# Autodesk Inventor assembly: Assembly Proximity Servo
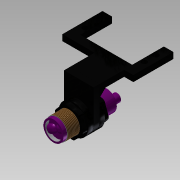
[picture p0: Inventor's stored thumbnail of the model, 180x180]
Saved by Autodesk Inventor 2015 SP1 (Build 190203100, 203)
## iProperties
Created: 2015-02-11
Part Number: Assembly Proximity Servo
Document SubType Name: Assembly
Designer: Rafi Kurnia Putra
Author: Rafi Kurnia Putra
## Documents named in this file (4)
- D:\Dropbox\krpai berkaki trui 2015\ROBUSTA\MEKANIK\ROBUSTA\Assembly Proximity Servo.iam
- D:\Dropbox\krpai berkaki trui 2015\ROBUSTA\MEKANIK\ROBUSTA\Dudukan Proximity Servo.ipt
- D:\Dropbox\krpai berkaki trui 2015\ROBUSTA\MEKANIK\ROBUSTA\Proximity.ipt
- D:\Dropbox\krpai berkaki trui 2015\ROBUSTA\MEKANIK\ROBUSTA\Proximity Gear.ipt
## Components (4 placed, 3 different names)
1. Dudukan Proximity Servo:1 — Mate:1, Mate:3, Flush:5, Mate:4, Mate:5, Flush:6, Mate:8
2. Proximity:1 — Mate:1, Mate:2, Mate:7, Flush:6
3. Proximity Gear:1 — Mate:2, Mate:3
4. Proximity Gear:2 — Mate:7, Mate:8
## Relationships (9: Mate 7, Flush 2)
- Mate:1: Dudukan Proximity Servo:1 ↔ Proximity:1
- Mate:2: Proximity:1 ↔ Proximity Gear:1
- Mate:3: Dudukan Proximity Servo:1 ↔ Proximity Gear:1
- Flush:5: Dudukan Proximity Servo:1
- Mate:4: Dudukan Proximity Servo:1
- Mate:5: Dudukan Proximity Servo:1
- Mate:7: Proximity:1 ↔ Proximity Gear:2
- Flush:6 (18.311 mm): Dudukan Proximity Servo:1 ↔ Proximity:1
- Mate:8: Dudukan Proximity Servo:1 ↔ Proximity Gear:2
